# Autodesk Inventor assembly: Assem6speedgearbox
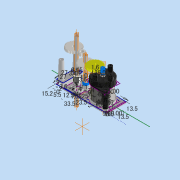
[picture p0: Inventor's stored thumbnail of the model, 180x180]
Saved by Autodesk Inventor 2022 (Build 260153000, 153)
## iProperties
Created: 2024-04-23
Part Number: Assem6speedgearbox
Document SubType Name: Assembly
Designer: ktamu
Author: ktamu
## Documents named in this file (13)
- D:\SDinventor\GearBox6Speed\Assem6speedgearbox.iam
- D:\SDinventor\GearBox6Speed\B1cover.ipt
- D:\SDinventor\GearBox6Speed\B3board.ipt
- D:\SDinventor\GearBox6Speed\driveshaft.ipt
- D:\SDinventor\GearBox6Speed\shaft4x45.ipt
- D:\SDinventor\GearBox6Speed\GearHub6kakku.ipt
- D:\SDinventor\GearBox6Speed\G9hub.ipt
- D:\SDinventor\GearBox6Speed\motor_for6speedgearbox.ipt
- D:\SDinventor\GearBox6Speed\motorshaft2x38.ipt
- D:\SDinventor\GearBox6Speed\Assem6speedgearbox\デザイン アクセラレータ\平歯車autoB1.iam
- D:\SDinventor\GearBox6Speed\Assem6speedgearbox\デザイン アクセラレータ\auto8-36g111.iam
- D:\SDinventor\GearBox6Speed\B4board.ipt
- D:\SDinventor\GearBox6Speed\Assem6speedgearbox\デザイン アクセラレータ\auto14-36g7andYell1.iam
## Components (12 placed, 12 different names)
1. B1cover:1 — 挿入:8, 回転:3, 挿入:12
2. B3board:1 — 挿入:2, 挿入:4, メイト:1, 挿入:6, 角度:1, 挿入:9, 挿入:10
3. driveshaft:1 — 挿入:2, 挿入:3, 回転:1
4. shaft4x45:1 — 挿入:4, 挿入:5, 回転:2
5. GearHub6kakku:1 — 挿入:3, 回転:1
6. G9hub:1 — 挿入:5, 回転:2, 挿入:14
7. motor_for6speedgearbox:1 — メイト:1, 挿入:6, 角度:1, 挿入:7, 挿入:8, 回転:3, 挿入:13
8. motorshaft2x38:1 — 挿入:7
9. auto8-36g11:1 [sub-assembly] — メイト:2, フラッシュ:1, 挿入:11, 挿入:13, 回転:4
10. auto14-36g7andYell:1 [sub-assembly] — 挿入:11, 挿入:12, 挿入:14, 回転:4
11. B4board:1 — 挿入:9, 挿入:10
12. auto14-36g7andBlue:1 [sub-assembly]
## Relationships (21: Insert 13, RelateRotation 4, Mate 2, Angle 1, Flush 1)
- 挿入:2 [Insert] (-26 mm): B3board:1 ↔ driveshaft:1
- 挿入:3 [Insert] (-46 mm): driveshaft:1 ↔ GearHub6kakku:1
- 回転:1 [RelateRotation] (1 ul): driveshaft:1 ↔ GearHub6kakku:1
- 挿入:4 [Insert] (-11.3 mm): B3board:1 ↔ shaft4x45:1
- 挿入:5 [Insert] (31 mm): shaft4x45:1 ↔ G9hub:1
- 回転:2 [RelateRotation] (1 ul): shaft4x45:1 ↔ G9hub:1
- メイト:1 [Mate]: B3board:1 ↔ motor_for6speedgearbox:1
- 挿入:6 [Insert]: B3board:1 ↔ motor_for6speedgearbox:1
- 角度:1 [Angle] (0 deg): B3board:1 ↔ motor_for6speedgearbox:1
- 挿入:7 [Insert] (-6.9 mm): motor_for6speedgearbox:1 ↔ motorshaft2x38:1
- 挿入:8 [Insert]: B1cover:1 ↔ motor_for6speedgearbox:1
- 回転:3 [RelateRotation] (1 ul): B1cover:1 ↔ motor_for6speedgearbox:1
- メイト:2 [Mate]: auto8-36g11:1
- フラッシュ:1 [Flush]: auto8-36g11:1
- 挿入:9 [Insert]: B3board:1 ↔ B4board:1
- 挿入:10 [Insert]: B3board:1 ↔ B4board:1
- 挿入:11 [Insert]: auto8-36g11:1 ↔ auto14-36g7andYell:1
- 挿入:12 [Insert]: B1cover:1 ↔ auto14-36g7andYell:1
- 挿入:13 [Insert] (1.54 mm): motor_for6speedgearbox:1 ↔ auto8-36g11:1
- 挿入:14 [Insert] (19.84 mm): G9hub:1 ↔ auto14-36g7andYell:1
- 回転:4 [RelateRotation] (1 ul): auto8-36g11:1 ↔ auto14-36g7andYell:1
